# Autodesk Inventor assembly: 537123 ADNGF-12-50-P-A---(0)
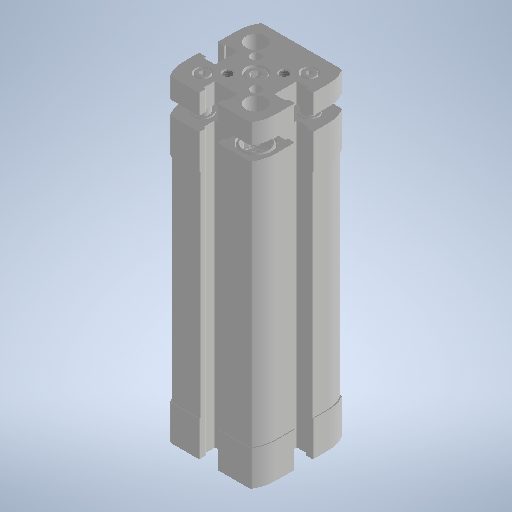
[picture p0: Inventor's stored thumbnail of the model, 512x512]
Saved by Autodesk Inventor 2025.2 (Build 292293000, 293)
## iProperties
Category: PARTsolutions
Company: FESTO
Created: 2025-06-09
Part Number: 537123 ADNGF-12-50-P-A---(0)
Catalog Web Link: www.cadenas.de
Description: ADNGF (m)-Compact cylinder, Modular system
Vendor: FESTO
Document SubType Name: Assembly
Designer: psAdmin
Manufacturer: FESTO
Mass: 146 g
Surface Area: 279.659 cm^2
Volume: 47.8189 cm^3
PSOL_IDENT_0: {ATYP=ASSISTANT},{DATA=script=$CADENAS_DATA/23d-libs/festo/webfesto.vbb&M_FAMILY=ADNGF&M_GROUP=01&M_
PSOL_IDENT_1: PARTNO=537123&IDCODE1=ADNGF-12-50-P-A&IDCODE2=&C_ADNGF_AF=A&C_ADNGF_DA=P&C_ADNGF_DM=12&C_ADNGF_HEAD=
PSOL_IDENT_2: ADNGF&HUB=50&NH_ADNGF_HUB=50&customer_number_cns=&MATES=1&LOD=HI&LOCKERP=1}
NB: 537123 ADNGF-12-50-P-A---(0)
NN: ADNGF (m)
NT: Compact cylinder, Modular system
NBSYN: $TNR. $TYP.-$HUB.-$DF.-$GA.$S2N.$S6N.$TLN.$ATEXN.---($HUBST.)
LINA: 537123 ADNGF-12-50-P-A
CATALOG: Festo
OFFICIAL_STANDARD_NUMBERS: ISO 21287
TNR: 537123
TYP: ADNGF-12
KDM: 12
HUB: 50
DF: P
GA: A
S2: -
S6: -
TL: -
ATEX: -
HUBST: 0
AF: 8
BG: 17
D1: 9
D4: 12
D5: 6
D6: M3
D7: 0
E: 27.5
EE: M5
FB: 3
G: 10.5
J2: 2
J3: 0
KF: M3
LA: 3.5
ME: 6
MM: 6
PL: 6
RT: M4
SF: 5
T1: 0
T2: 2.1
T4: 1.5
TG: 16
WH: 4.2
ZA: 35
ZB: 39.2
ZB2: 0
ZM: 44.5
ZM2: 0
CNSMASSEXACT: 0.146
SUPPLIER: FESTO
ARTICLENO: 537123 ADNGF-12-50-P-A---(0)
BOMINFO: 537123 ADNGF-12-50-P-A
CREATOR: CADENAS GmbH
Title: 537123 ADNGF-12-50-P-A
Author: Cadenas PARTsolutions
Comments: Compact cylinder, Modular system
## Documents named in this file (3)
- C:\Users\Jakob\Documents\Kooperatives Studium HHN\Studium\3. Semester\CAD_Konstruktion - Paspa\05_Useless_Box\CAD-Paspa\Useless Box\Eigene Bauteile\Greifer_Unterlegscheibe\Kaufteile\Führungszylinder\AIS2024\537123 ADNGF-12-50-P-A---(0).iam
- C:\Users\Jakob\Documents\Kooperatives Studium HHN\Studium\3. Semester\CAD_Konstruktion - Paspa\05_Useless_Box\CAD-Paspa\Useless Box\Eigene Bauteile\Greifer_Unterlegscheibe\Kaufteile\Führungszylinder\AIS2024\537123 ADNGF-12-50-P-A---(Z).ipt
- C:\Users\Jakob\Documents\Kooperatives Studium HHN\Studium\3. Semester\CAD_Konstruktion - Paspa\05_Useless_Box\CAD-Paspa\Useless Box\Eigene Bauteile\Greifer_Unterlegscheibe\Kaufteile\Führungszylinder\AIS2024\537123 ADNGF-12-50-P-A---(KS).ipt
## Components (2 placed, 2 different names)
1. 537123 ADNGF-12-50-P-A---(Z):1 — CYLINDER_XY@1 <-> PISTON_XY@2, CYLINDER_Z@1 <-> PISTON_Z@2, CYLINDER_YZ@1 <-> PISTON_YZ@2
2. 537123 ADNGF-12-50-P-A---(KS):1 — CYLINDER_XY@1 <-> PISTON_XY@2, CYLINDER_Z@1 <-> PISTON_Z@2, CYLINDER_YZ@1 <-> PISTON_YZ@2
## Relationships (3: Mate 2, Angle 1)
- CYLINDER_XY@1 <-> PISTON_XY@2 [Mate]: 537123 ADNGF-12-50-P-A---(Z):1 ↔ 537123 ADNGF-12-50-P-A---(KS):1
- CYLINDER_Z@1 <-> PISTON_Z@2 [Mate]: 537123 ADNGF-12-50-P-A---(Z):1 ↔ 537123 ADNGF-12-50-P-A---(KS):1
- CYLINDER_YZ@1 <-> PISTON_YZ@2 [Angle] (0 deg): 537123 ADNGF-12-50-P-A---(Z):1 ↔ 537123 ADNGF-12-50-P-A---(KS):1
